# Autodesk Inventor assembly: Cover_v3_v2_assy
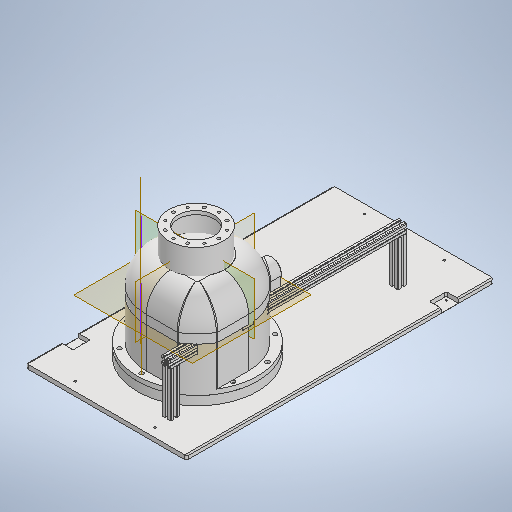
[picture p0: Inventor's stored thumbnail of the model, 512x512]
Saved by Autodesk Inventor 2025 (Build 290162000, 162)
## iProperties
Created: 2025-08-19
Part Number: Cover_v3_v2_assy
Document SubType Name: Assembly
Designer: mumin
Author: mumin
## Documents named in this file (9)
- C:\GitHub\In-situ-monitoring-of-powder-bed-fusion-additive-manufacturing\system_development\Orichalcum\v0.3\Cover_v3_v2_assy.iam
- C:\GitHub\In-situ-monitoring-of-powder-bed-fusion-additive-manufacturing\system_development\Orichalcum\v0.3\12mm Cover.ipt
- C:\GitHub\In-situ-monitoring-of-powder-bed-fusion-additive-manufacturing\system_development\Orichalcum\v0.3\SealedGlassRing.ipt
- C:\GitHub\In-situ-monitoring-of-powder-bed-fusion-additive-manufacturing\system_development\Orichalcum\v0.3\Cylinder Housing_base_2.ipt
- C:\GitHub\In-situ-monitoring-of-powder-bed-fusion-additive-manufacturing\system_development\Orichalcum\v0.3\Cover v3 Assembly\2020 Legs (100mm).ipt
- C:\GitHub\In-situ-monitoring-of-powder-bed-fusion-additive-manufacturing\system_development\Orichalcum\v0.3\Cover v3 Assembly\2020 LV-GVS Beam (530).ipt
- C:\GitHub\In-situ-monitoring-of-powder-bed-fusion-additive-manufacturing\system_development\Orichalcum\v0.3\Cylinder Housing_cap_2.ipt
- C:\GitHub\In-situ-monitoring-of-powder-bed-fusion-additive-manufacturing\system_development\Orichalcum\v0.3\Original Center Cylinder.ipt
- C:\GitHub\In-situ-monitoring-of-powder-bed-fusion-additive-manufacturing\system_development\Adamant\v0.1\hardware design\Cylinder Segment Camera Only.ipt
## Components (8 placed, 7 different names)
1. 12mm Cover:1 — Insert:1, Insert:2, Insert:5, Insert:6
2. SealedGlassRing:1 — Insert:1, Insert:2, Insert:3, Insert:4
3. Cylinder Housing_base_2:1 — Insert:3, Insert:4, Insert:7
4. 2020 Legs (100mm):1 — Insert:5, Mate:1, Flush:1, Flush:2
5. 2020 Legs (100mm):2 — Insert:6
6. 2020 LV-GVS Beam (530):1 — Mate:1, Flush:1, Flush:2
7. Cylinder Housing_cap_2:1 — Insert:7
8. Original Center Cylinder:1
## Relationships (10: Insert 7, Flush 2, Mate 1)
- Insert:1: 12mm Cover:1 ↔ SealedGlassRing:1
- Insert:2: 12mm Cover:1 ↔ SealedGlassRing:1
- Insert:3: SealedGlassRing:1 ↔ Cylinder Housing_base_2:1
- Insert:4: SealedGlassRing:1 ↔ Cylinder Housing_base_2:1
- Insert:5: 12mm Cover:1 ↔ 2020 Legs (100mm):1
- Insert:6: 12mm Cover:1 ↔ 2020 Legs (100mm):2
- Mate:1: 2020 Legs (100mm):1 ↔ 2020 LV-GVS Beam (530):1
- Flush:1: 2020 Legs (100mm):1 ↔ 2020 LV-GVS Beam (530):1
- Flush:2: 2020 Legs (100mm):1 ↔ 2020 LV-GVS Beam (530):1
- Insert:7: Cylinder Housing_base_2:1 ↔ Cylinder Housing_cap_2:1
